# Autodesk Inventor assembly: 900-50-PROFILES-ANGLE-CONN-30x30-01
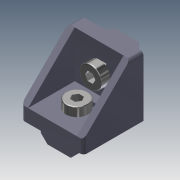
[picture p0: Inventor's stored thumbnail of the model, 180x180]
Saved by Autodesk Inventor 2018.2 (Build 222227000, 227)
## iProperties
Manager: feesmrt
Company: FRANCOR
Created: 2017-12-16
Part Number: 900-50-PROFILES-ANGLE-CONN-30x30-01
Material: Generisch
Document SubType Name: Assembly
Designer: feesmrt
Project: Rescue Robot
Cost Center: -
Description: Rocker Bearing 30 Profile Connector ASM
Engineer: feesmrt
Authority: feesmrt
Stock Number: 900-50-PROFILES-ANGLE-CONN-30x30-01
Author: feesmrt
Title: Rocker Bearing 30 Profile Connector ASM
Subject: Rescue Robot
Revision Number: 1
## Documents named in this file (4)
- D:\Programmierung\FRANC0R\CAD\02-Rocker-Bogie-Robot\900-COMPONENTS\900-50-PROFILES\900-50-PROFILES-ANGLE-CONN-30x30-01.iam
- D:\Programmierung\FRANC0R\CAD\02-Rocker-Bogie-Robot\900-COMPONENTS\900-50-PROFILES\900-50-PROFILES-ANGLE-CONN-30x30.ipt
- D:\Programmierung\FRANC0R\CAD\02-Rocker-Bogie-Robot\900-COMPONENTS\900-40-SCREWS\900-40-SCREWS-DIN7984_M6x12.ipt
- D:\Programmierung\FRANC0R\CAD\02-Rocker-Bogie-Robot\900-COMPONENTS\900-50-PROFILES\900-50-PROFILES-CONN-N8xM6.ipt
## Components (5 placed, 3 different names)
1. 900-50-PROFILES-ANGLE-CONN-30x30:1 — Passend:3, Passend:4, Passend:5, Passend:7, Passend:8, Passend:9, Winkel:1, Passend:10, Passend:12
2. 900-40-SCREWS-DIN7984_M6x12:1 — Passend:3, Passend:4, Passend:5, Passend:6
3. 900-50-PROFILES-CONN-N8xM6:1 — Passend:6, Passend:7, Passend:8
4. 900-40-SCREWS-DIN7984_M6x12:2 — Passend:9, Winkel:1, Passend:10, Fluchtend:1, Passend:11
5. 900-50-PROFILES-CONN-N8xM6:2 — Passend:11, Passend:12, Passend:13
## Relationships (13: Mate 11, Angle 1, Flush 1)
- Passend:3 [Mate]: 900-50-PROFILES-ANGLE-CONN-30x30:1 ↔ 900-40-SCREWS-DIN7984_M6x12:1
- Passend:4 [Mate]: 900-50-PROFILES-ANGLE-CONN-30x30:1 ↔ 900-40-SCREWS-DIN7984_M6x12:1
- Passend:5 [Mate] (-16 mm): 900-50-PROFILES-ANGLE-CONN-30x30:1 ↔ 900-40-SCREWS-DIN7984_M6x12:1
- Passend:6 [Mate]: 900-40-SCREWS-DIN7984_M6x12:1 ↔ 900-50-PROFILES-CONN-N8xM6:1
- Passend:7 [Mate] (2.8 mm): 900-50-PROFILES-ANGLE-CONN-30x30:1 ↔ 900-50-PROFILES-CONN-N8xM6:1
- Passend:8 [Mate]: 900-50-PROFILES-ANGLE-CONN-30x30:1 ↔ 900-50-PROFILES-CONN-N8xM6:1
- Passend:9 [Mate]: 900-50-PROFILES-ANGLE-CONN-30x30:1 ↔ 900-40-SCREWS-DIN7984_M6x12:2
- Winkel:1 [Angle] (0 deg): 900-50-PROFILES-ANGLE-CONN-30x30:1 ↔ 900-40-SCREWS-DIN7984_M6x12:2
- Passend:10 [Mate] (-15 mm): 900-50-PROFILES-ANGLE-CONN-30x30:1 ↔ 900-40-SCREWS-DIN7984_M6x12:2
- Fluchtend:1 [Flush]: 900-40-SCREWS-DIN7984_M6x12:2
- Passend:11 [Mate]: 900-40-SCREWS-DIN7984_M6x12:2 ↔ 900-50-PROFILES-CONN-N8xM6:2
- Passend:12 [Mate] (2.8 mm): 900-50-PROFILES-ANGLE-CONN-30x30:1 ↔ 900-50-PROFILES-CONN-N8xM6:2
- Passend:13 [Mate]: 900-50-PROFILES-CONN-N8xM6:2
